# Autodesk Inventor assembly: CL4-200
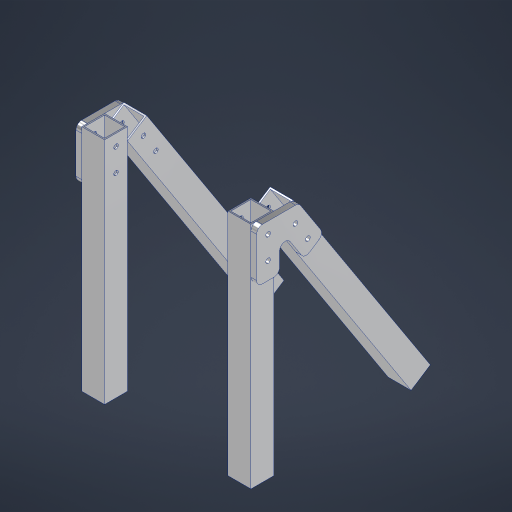
[picture p0: Inventor's stored thumbnail of the model, 512x512]
Saved by Autodesk Inventor 2023.4 (Build 274418000, 418)
## iProperties
Created: 2025-02-04
Part Number: CL4-200
Document SubType Name: Assembly
Designer: brand
Author: brand
## Documents named in this file (4)
- C:\Users\brand\OneDrive\Documents\GitHub\robotics 23\2025-ReefScape---CAD\Climber\CL4\CL4-200.iam
- C:\Users\brand\OneDrive\Documents\GitHub\robotics 23\2025-ReefScape---CAD\Climber\CL4\CL4-002.ipt
- C:\Users\brand\OneDrive\Documents\GitHub\robotics 23\2025-ReefScape---CAD\Climber\CL4\CL4-007.ipt
- C:\Users\brand\OneDrive\Documents\GitHub\robotics 23\2025-ReefScape---CAD\Climber\CL4\CL4-009.ipt
## Components (6 placed, 3 different names)
1. CL4-002:1 — Flush:1, Flush:2, Insert:1, Insert:2
2. CL4-002:2 — Flush:1, Flush:2, Insert:5, Insert:6
3. CL4-007:1 — Insert:7, Insert:8
4. CL4-007:2 — Insert:3, Insert:4
5. CL4-009:1 — Insert:1, Insert:2, Insert:3, Insert:4
6. CL4-009:2 — Insert:5, Insert:6, Insert:7, Insert:8
## Relationships (10: Insert 8, Flush 2)
- Flush:1: CL4-002:1 ↔ CL4-002:2
- Flush:2: CL4-002:1 ↔ CL4-002:2
- Insert:1: CL4-002:1 ↔ CL4-009:1
- Insert:2: CL4-002:1 ↔ CL4-009:1
- Insert:3: CL4-007:2 ↔ CL4-009:1
- Insert:4: CL4-007:2 ↔ CL4-009:1
- Insert:5: CL4-002:2 ↔ CL4-009:2
- Insert:6: CL4-002:2 ↔ CL4-009:2
- Insert:7: CL4-007:1 ↔ CL4-009:2
- Insert:8: CL4-007:1 ↔ CL4-009:2
